# Autodesk Inventor assembly: 足首_独立ピッチ_1
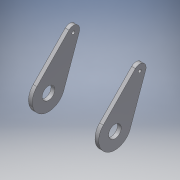
[picture p0: Inventor's stored thumbnail of the model, 180x180]
Saved by Autodesk Inventor 2018 (Build 220112000, 112)
## iProperties
Created: 2016-05-04
Part Number: 足首_独立ピッチ_1
Document SubType Name: Assembly
Designer: hiroaki
Mass: 12.4515 g
Surface Area: 78.9605 cm^2
Volume: 4.53639 cm^3
Density: 2.74481 g/cm^3
Author: hiroaki
## Documents named in this file (2)
- C:\Users\taka\Desktop\OPR\OpenPlatform_ver1_0\下半身\足首\足首_独立ピッチ_1.iam
- C:\Users\taka\Desktop\OPR\OpenPlatform_ver1_0\下半身\足首\足首_独立ピッチ_1_1.ipt
## Components (2 placed, 1 different names)
1. 足首_独立ピッチ_1_1:1 — メイト:2, メイト:5, メイト:6
2. 足首_独立ピッチ_1_1:2 — メイト:2, メイト:6, 角度:1
## Relationships (4: Mate 3, Angle 1)
- メイト:2 [Mate] (50.3 mm): 足首_独立ピッチ_1_1:1 ↔ 足首_独立ピッチ_1_1:2
- メイト:5 [Mate] (25.15 mm): 足首_独立ピッチ_1_1:1
- メイト:6 [Mate]: 足首_独立ピッチ_1_1:1 ↔ 足首_独立ピッチ_1_1:2
- 角度:1 [Angle] (0 deg): 足首_独立ピッチ_1_1:2
